# Autodesk Inventor assembly: wallMountTop
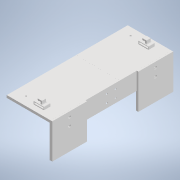
[picture p0: Inventor's stored thumbnail of the model, 180x180]
Saved by Autodesk Inventor 2021 (Build 250183000, 183)
## iProperties
Created: 2021-02-26
Part Number: wallMountTop
Document SubType Name: Assembly
Designer: jjaken
Author: jjaken
## Documents named in this file (4)
- C:\Users\jjaken\git\github\CAD-Projects\catPerchHolder\wallMountTop.iam
- C:\Users\jjaken\git\github\CAD-Projects\catPerchHolder\leftTop.ipt
- C:\Users\jjaken\git\github\CAD-Projects\catPerchHolder\rightTop.ipt
- C:\Users\jjaken\git\github\CAD-Projects\catPerchHolder\wallMountBottom.ipt
## Components (4 placed, 3 different names)
1. leftTop:1 — Mate:1, Mate:2, Mate:3
2. rightTop:1 — Mate:4, Mate:5, Mate:6
3. wallMountBottom:1 — Mate:4, Mate:5, Mate:6
4. wallMountBottom:2 — Mate:1, Mate:2, Mate:3
## Relationships (6: Mate 6)
- Mate:1: leftTop:1 ↔ wallMountBottom:2
- Mate:2: leftTop:1 ↔ wallMountBottom:2
- Mate:3: leftTop:1 ↔ wallMountBottom:2
- Mate:4: rightTop:1 ↔ wallMountBottom:1
- Mate:5: rightTop:1 ↔ wallMountBottom:1
- Mate:6: rightTop:1 ↔ wallMountBottom:1
